# Autodesk Inventor assembly: Truss
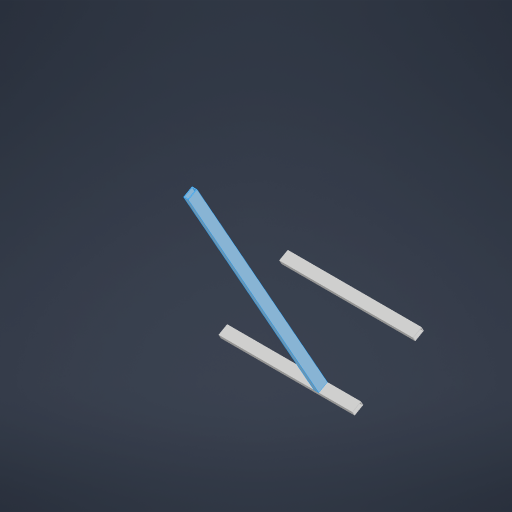
[picture p0: Inventor's stored thumbnail of the model, 512x512]
Saved by Autodesk Inventor 2023 (Build 270158000, 158)
## iProperties
Created: 2023-01-10
Part Number: Truss
Document SubType Name: Assembly
Designer: Terrence
Mass: 9567.53 g
Surface Area: 21493.6 cm^2
Volume: 3543.53 cm^3
Density: 2.7 g/cm^3
Author: Terrence
## Documents named in this file (3)
- C:\Users\Terrence\Documents\FRC Long\Truss\Truss.iam
- C:\Users\Terrence\Documents\FRC Long\Truss\Solid1_1.ipt
- C:\Users\Terrence\Documents\FRC Long\Truss\Solid3_1.ipt
## Components (3 placed, 2 different names)
1. Solid3_1:1 — Flush:13, Mate:11, Flush:14
2. Solid1_1:3 — Flush:13, Mate:11, Flush:14
3. Solid3_1:2
## Relationships (3: Flush 2, Mate 1)
- Flush:13: Solid3_1:1 ↔ Solid1_1:3
- Mate:11: Solid3_1:1 ↔ Solid1_1:3
- Flush:14 (171.45 mm): Solid3_1:1 ↔ Solid1_1:3
